# Autodesk Inventor assembly: Assembly1
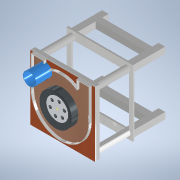
[picture p0: Inventor's stored thumbnail of the model, 180x180]
Saved by Autodesk Inventor 2021 (Build 250183000, 183)
## iProperties
Created: 2021-07-27
Part Number: Assembly1
Document SubType Name: Assembly
Designer: user
Author: user
## Documents named in this file (6)
- E:\cannon\FRISBEE LAUNCHER\Assembly1.iam
- E:\cannon\tABLE.ipt
- E:\cannon\FRISBEE LAUNCHER\base.ipt
- E:\cannon\FRISBEE LAUNCHER\new wheel.ipt
- E:\cannon\FRISBEE LAUNCHER\cyan frisbee holder.ipt
- E:\cannon\FRISBEE LAUNCHER\frisbeeeeeeee.ipt
## Components (5 placed, 5 different names)
1. tABLE:1 — Mate:1, Rigid:1, Angle:1
2. base:1 — Mate:1, Rigid:1, Rigid:2, Mate:2
3. cyan frisbee holder:1 — Rigid:2
4. frisbeeeeeeee:2
5. new wheel:1 — Mate:2, Angle:1
## Relationships (5: Mate 2, WeldJoint 2, Angle 1)
- Mate:1: tABLE:1 ↔ base:1
- Rigid:1 [WeldJoint]: tABLE:1 ↔ base:1
- Rigid:2 [WeldJoint]: base:1 ↔ cyan frisbee holder:1
- Mate:2: base:1 ↔ new wheel:1
- Angle:1 (0 deg): tABLE:1 ↔ new wheel:1
